# Autodesk Inventor assembly: 000ASS_Bo_banh_xe_02
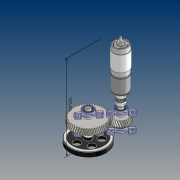
[picture p0: Inventor's stored thumbnail of the model, 180x180]
Saved by Autodesk Inventor 2021 (Build 250183000, 183)
## iProperties
Created: 2024-03-11
Part Number: 000ASS_Bo_banh_xe_02
Document SubType Name: Assembly
Designer: Admin
Author: Admin
## Documents named in this file (9)
- C:\Users\Admin\Desktop\DO_AN_TOT_NGHIEP_2024\Mechanical\Design_in_3D\Version_1\000ASS_Bo_banh_xe_02.iam
- C:\Users\Admin\Desktop\DO_AN_TOT_NGHIEP_2024\Mechanical\Design_in_3D\Version_1\01_Truc_01.ipt
- C:\Users\Admin\Desktop\DO_AN_TOT_NGHIEP_2024\Mechanical\Design_in_3D\Library\kp08-baering-with-housing-1.snapshot.4\KP08.iam
- C:\Users\Admin\Desktop\DO_AN_TOT_NGHIEP_2024\Mechanical\Design_in_3D\Library\planetary-gear-dc-motor-2.snapshot.1\Planetary Gear DC Motor\Planatary motor v1.ipt
- C:\Users\Admin\Desktop\DO_AN_TOT_NGHIEP_2024\Mechanical\Design_in_3D\Library\kh-p-n-i-m-m-2.snapshot.1\khop-noi-mem.ipt
- C:\Users\Admin\Desktop\DO_AN_TOT_NGHIEP_2024\Mechanical\Design_in_3D\Library\banh-xe-robot-nhom-v5_2-1.snapshot.1\95mm phi 8 99g.ipt
- C:\Users\Admin\Desktop\DO_AN_TOT_NGHIEP_2024\Mechanical\Design_in_3D\Version_1\02_Truc_01.ipt
- C:\Users\Admin\Desktop\DO_AN_TOT_NGHIEP_2024\Mechanical\Design_in_3D\Version_1\03_Banh_rang_bi_dan_1.ipt
- C:\Users\Admin\Desktop\DO_AN_TOT_NGHIEP_2024\Mechanical\Design_in_3D\Version_1\04_Banh_rang_dan_1.ipt
## Components (11 placed, 8 different names)
1. 01_Truc_01:1 — Mate:1, Mate:2, Mate:3, Flush:2, Mate:11, Mate:13
2. KP08:1 [sub-assembly] — Mate:2, Flush:1, Flush:6, Mate:17
3. KP08:2 [sub-assembly] — Mate:3, Flush:1, Flush:2, Flush:4, Flush:5, Mate:15
4. Planatary motor v1:1 — Mate:1, Mate:5
5. khop-noi-mem:1 — Mate:5, Mate:17, Rotation:4
6. KP08:3 [sub-assembly] — Flush:4, Flush:5, Mate:10, Flush:10, Mate:16, Angle:1
7. KP08:4 [sub-assembly] — Flush:6, Flush:7, Flush:10, Mate:14
8. 95mm phi 8 99g:1 — Mate:10, Flush:8, Rotation:2
9. 02_Truc_01:1 — Flush:7, Flush:8, Mate:12, Mate:13, Mate:14, Mate:16
10. Spur Gear2:1 — Mate:12, Flush:9, Rotation:2, Angle:1, Rotation:3
11. Spur Gear1:1 — Mate:11, Flush:9, Mate:15, Rotation:3, Rotation:4
## Relationships (25: Mate 12, Flush 9, RelateRotation 3, Angle 1)
- Mate:1: 01_Truc_01:1 ↔ Planatary motor v1:1
- Mate:2: 01_Truc_01:1 ↔ KP08:1
- Mate:3: 01_Truc_01:1 ↔ KP08:2
- Flush:1: KP08:1 ↔ KP08:2
- Flush:2: 01_Truc_01:1 ↔ KP08:2
- Mate:5: Planatary motor v1:1 ↔ khop-noi-mem:1
- Flush:4: KP08:2 ↔ KP08:3
- Flush:5: KP08:2 ↔ KP08:3
- Flush:6: KP08:1 ↔ KP08:4
- Mate:10: KP08:3 ↔ 95mm phi 8 99g:1
- Flush:7: KP08:4 ↔ 02_Truc_01:1
- Flush:8: 95mm phi 8 99g:1 ↔ 02_Truc_01:1
- Mate:11: 01_Truc_01:1 ↔ Spur Gear1:1
- Mate:12: 02_Truc_01:1 ↔ Spur Gear2:1
- Flush:9: Spur Gear2:1 ↔ Spur Gear1:1
- Mate:13 (60 mm): 01_Truc_01:1 ↔ 02_Truc_01:1
- Flush:10: KP08:3 ↔ KP08:4
- Mate:14: KP08:4 ↔ 02_Truc_01:1
- Mate:15 (5 mm): KP08:2 ↔ Spur Gear1:1
- Mate:16: KP08:3 ↔ 02_Truc_01:1
- Mate:17 (5 mm): KP08:1 ↔ khop-noi-mem:1
- Rotation:2 [RelateRotation] (1 ul): 95mm phi 8 99g:1 ↔ Spur Gear2:1
- Angle:1 (1014 deg): KP08:3 ↔ Spur Gear2:1
- Rotation:3 [RelateRotation] (0.5 ul): Spur Gear2:1 ↔ Spur Gear1:1
- Rotation:4 [RelateRotation] (1 ul): khop-noi-mem:1 ↔ Spur Gear1:1
